# Autodesk Inventor assembly: Leg_Right_v1_MIR
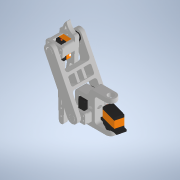
[picture p0: Inventor's stored thumbnail of the model, 180x180]
Saved by Autodesk Inventor 2020.3 (Build 243373000, 373)
## iProperties
Created: 2021-03-06
Part Number: Leg_Right_v1_MIR
Document SubType Name: Assembly
Designer: sanyi
Author: sanyi
## Documents named in this file (6)
- C:\Users\sanyi\Documents\Inventor\Quadropod\Leg_Right_v1_MIR.iam
- C:\Users\sanyi\Documents\Inventor\Quadropod\LegStart_v1_MIR.ipt
- C:\Users\sanyi\Documents\Inventor\Quadropod\LegEnd_Right_v1_MIR.ipt
- C:\Users\sanyi\Documents\Inventor\Quadropod\LegMiddle_Final_1_MIR.ipt
- C:\Users\sanyi\Documents\Inventor\Quadropod\LegPin_v1_MIR.ipt
- C:\Users\sanyi\Documents\Inventor\Quadropod\SH-0257MG_MIR.ipt
## Components (8 placed, 5 different names)
1. LegStart_v1_MIR:1 — Flush:1, Mate:11, Mate:10, Insert:9, Insert:8, Mate:8, Insert:10, Angle:1, Mate:4, Mate:7, Mate:6
2. LegEnd_Right_v1_MIR:1 — Insert:12, Insert:11, Mate:9, Mate:2, Angle:2, Insert:7, Mate:5
3. LegMiddle_Final_1_MIR:1 — Insert:13, Insert:6
4. LegPin_v1_MIR:1 — Insert:13, Insert:9, Insert:8, Mate:8
5. LegPin_v1_MIR:2 — Insert:12, Insert:11, Mate:9, Insert:6, Mate:2
6. SH-0257MG_MIR:1 — Insert:10, Angle:1, Mate:4
7. SH-0257MG_MIR:2 — Mate:7, Mate:6
8. SH-0257MG_MIR:3 — Angle:2, Insert:7, Mate:5
## Relationships (20: Mate 8, Insert 8, Flush 2, Angle 2)
- Flush:1: LegStart_v1_MIR:1
- Mate:11: LegStart_v1_MIR:1
- Mate:10 [Flush]: LegStart_v1_MIR:1
- Insert:13 (0.2 mm): LegMiddle_Final_1_MIR:1 ↔ LegPin_v1_MIR:1
- Insert:9: LegStart_v1_MIR:1 ↔ LegPin_v1_MIR:1
- Insert:8: LegStart_v1_MIR:1 ↔ LegPin_v1_MIR:1
- Mate:8: LegStart_v1_MIR:1 ↔ LegPin_v1_MIR:1
- Insert:12: LegEnd_Right_v1_MIR:1 ↔ LegPin_v1_MIR:2
- Insert:11: LegEnd_Right_v1_MIR:1 ↔ LegPin_v1_MIR:2
- Mate:9: LegEnd_Right_v1_MIR:1 ↔ LegPin_v1_MIR:2
- Insert:6 (0.2 mm): LegMiddle_Final_1_MIR:1 ↔ LegPin_v1_MIR:2
- Mate:2: LegEnd_Right_v1_MIR:1 ↔ LegPin_v1_MIR:2
- Insert:10: LegStart_v1_MIR:1 ↔ SH-0257MG_MIR:1
- Angle:1 (0 deg): LegStart_v1_MIR:1 ↔ SH-0257MG_MIR:1
- Mate:4: LegStart_v1_MIR:1 ↔ SH-0257MG_MIR:1
- Mate:7: LegStart_v1_MIR:1 ↔ SH-0257MG_MIR:2
- Mate:6: LegStart_v1_MIR:1 ↔ SH-0257MG_MIR:2
- Angle:2 (0 deg): LegEnd_Right_v1_MIR:1 ↔ SH-0257MG_MIR:3
- Insert:7: LegEnd_Right_v1_MIR:1 ↔ SH-0257MG_MIR:3
- Mate:5: LegEnd_Right_v1_MIR:1 ↔ SH-0257MG_MIR:3
